# Autodesk Inventor assembly: worm
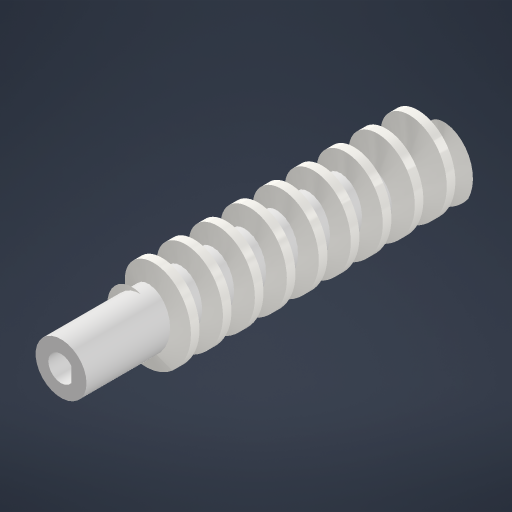
[picture p0: Inventor's stored thumbnail of the model, 512x512]
Saved by Autodesk Inventor 2024 (Build 280153000, 153)
## iProperties
Created: 2023-06-18
Part Number: worm
Document SubType Name: Assembly
Designer: 6gioc
Mass: 59.4569 g
Surface Area: 70.2749 cm^2
Volume: 11.1989 cm^3
Density: 5.30915 g/cm^3
Author: 6gioc
## Documents named in this file (3)
- C:\Users\6gioc\OneDrive\AAST\PART\worm.iam
- C:\Users\6gioc\OneDrive\AAST\PART\base worm.ipt
- C:\Users\6gioc\OneDrive\AAST\PART\worm\디자인 액셀러레이터\웜 기어1.iam
## Components (2 placed, 2 different names)
1. base worm:1 — 메이트:1, 각도:1
2. 웜 기어:1 [sub-assembly] — 메이트:1, 각도:1
## Relationships (2: Mate 1, Angle 1)
- 메이트:1 [Mate]: base worm:1 ↔ 웜 기어:1
- 각도:1 [Angle] (0 deg): base worm:1 ↔ 웜 기어:1
